# Autodesk Inventor assembly: Assembly1
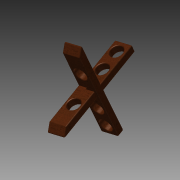
[picture p0: Inventor's stored thumbnail of the model, 180x180]
Saved by Autodesk Inventor 2015 (Build 190159000, 159)
## iProperties
Created: 2014-07-27
Part Number: Assembly1
Document SubType Name: Assembly
Designer: pc
Author: pc
## Documents named in this file (2)
- C:\Users\pc\Documents\blinds\openscad\sunil\Assembly1.iam
- C:\Users\pc\Documents\blinds\openscad\sunil\stand1.ipt
## Components (2 placed, 1 different names)
1. stand1:1 — Mate:1, Mate:2
2. stand1:2 — Mate:1, Mate:2
## Relationships (2: Mate 2)
- Mate:1: stand1:1 ↔ stand1:2
- Mate:2: stand1:1 ↔ stand1:2
